# Autodesk Inventor assembly: Winch Concept
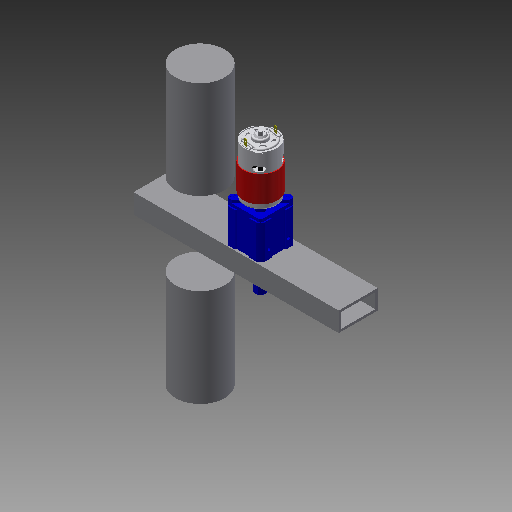
[picture p0: Inventor's stored thumbnail of the model, 512x512]
Saved by Autodesk Inventor 2018 (Build 220112000, 112)
## iProperties
Created: 2018-01-29
Part Number: Winch Concept
Document SubType Name: Assembly
Designer: Apple
Author: Apple
## Documents named in this file (4)
- C:\Users\Apple\Documents\Inventor\2018 PowerUp\Winch\Winch Concept.iam
- C:\Users\Apple\Documents\Inventor\2018 PowerUp\Winch\Winch Drum Concept.ipt
- C:\Users\Apple\Documents\Inventor\2018 PowerUp\AndyMark\Sport57 w Redline Motor 100_1.iam
- C:\Users\Apple\Documents\Inventor\2018 PowerUp\Winch\Motor Mount.ipt
## Components (4 placed, 3 different names)
1. Winch Drum Concept:1
2. Winch Drum Concept:2
3. Sport57 w Redline Motor 100_1:1 [sub-assembly] — Mate:2, Mate:3
4. Motor Mount:1 — Mate:2, Mate:3
## Relationships (3: Mate 3)
- [Mate]: Winch Drum Concept:1 ↔ Winch Drum Concept:2
- Mate:2: Sport57 w Redline Motor 100_1:1 ↔ Motor Mount:1
- Mate:3: Sport57 w Redline Motor 100_1:1 ↔ Motor Mount:1
